# Autodesk Inventor assembly: GFRP_T2_05
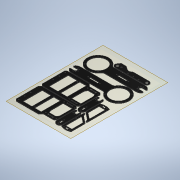
[picture p0: Inventor's stored thumbnail of the model, 180x180]
Saved by Autodesk Inventor 2020 (Build 240168000, 168)
## iProperties
Created: 2021-08-27
Part Number: GFRP_T2_05
Document SubType Name: Assembly
Designer: Masato
Author: Masato
## Documents named in this file (7)
- C:\Users\naoki\Documents\Inventor\CitBrains\git_clone\SUSTAINA_ver1_0\A_T2_175\SUSTAINA-OP\Cam\GFRP_T2_05.iam
- C:\Users\naoki\Documents\Inventor\CitBrains\git_clone\SUSTAINA_ver1_0\A_T2_175\SUSTAINA-OP\Cam\DisposableBoard.ipt
- C:\Users\naoki\Documents\Inventor\CitBrains\git_clone\SUSTAINA_ver1_0\A_T2_175\SUSTAINA-OP\UpperBody\Trunk\Trunk_upper_side_frame.ipt
- C:\Users\naoki\Documents\Inventor\CitBrains\git_clone\SUSTAINA_ver1_0\A_T2_175\SUSTAINA-OP\UpperBody\Arm\ForeArm_outside_frame.ipt
- C:\Users\naoki\Documents\Inventor\CitBrains\git_clone\SUSTAINA_ver1_0\A_T2_175\SUSTAINA-OP\UpperBody\Arm\UpperArm_side_frame.ipt
- C:\Users\naoki\Documents\Inventor\CitBrains\git_clone\SUSTAINA_ver1_0\A_T2_175\SUSTAINA-OP\UpperBody\Arm\ForeArm_inside_frame.ipt
- C:\Users\naoki\Documents\Inventor\CitBrains\git_clone\SUSTAINA_ver1_0\A_T2_175\SUSTAINA-OP\LowerBody\Link\BackLink_frame.ipt
## Components (10 placed, 6 different names)
1. DisposableBoard:1 — メイト:2, メイト:1, フラッシュ:1, フラッシュ:2, メイト:7, メイト:8, 正接:2, 正接:3, メイト:9, メイト:12, メイト:14, メイト:15, メイト:16, フラッシュ:3, フラッシュ:4, メイト:19, メイト:20, フラッシュ:6, 正接:6, 正接:7
2. Trunk_upper_side_frame:1 — メイト:15, フラッシュ:5, メイト:18, メイト:24, メイト:25
3. Trunk_upper_side_frame:2 — メイト:12, フラッシュ:3, フラッシュ:4, フラッシュ:5, メイト:18, メイト:21
4. ForeArm_outside_frame:1 — メイト:7, 正接:2, 正接:3, メイト:25, 正接:8, 正接:9
5. ForeArm_outside_frame:2 — メイト:8, メイト:17, 正接:7, 正接:8, 正接:9, 正接:10
6. UpperArm_side_frame:1 — メイト:9, メイト:23, 正接:4
7. ForeArm_inside_frame:1 — メイト:19, メイト:21, メイト:22, 正接:5, 正接:6
8. UpperArm_side_frame:2 — メイト:14, メイト:22, フラッシュ:6, 正接:4
9. ForeArm_inside_frame:2 — メイト:20, メイト:23, メイト:24, 正接:5
10. BackLink_frame:1 — メイト:16, メイト:17, 正接:10
## Relationships (33: Mate 18, Tangent 9, Flush 6)
- メイト:2 [Mate]: DisposableBoard:1
- メイト:1 [Mate]: DisposableBoard:1
- フラッシュ:1 [Flush]: DisposableBoard:1
- フラッシュ:2 [Flush]: DisposableBoard:1
- メイト:7 [Mate]: DisposableBoard:1 ↔ ForeArm_outside_frame:1
- メイト:8 [Mate]: DisposableBoard:1 ↔ ForeArm_outside_frame:2
- 正接:2 [Tangent] (2.5 mm): DisposableBoard:1 ↔ ForeArm_outside_frame:1
- 正接:3 [Tangent] (2.5 mm): DisposableBoard:1 ↔ ForeArm_outside_frame:1
- メイト:9 [Mate]: DisposableBoard:1 ↔ UpperArm_side_frame:1
- メイト:12 [Mate]: DisposableBoard:1 ↔ Trunk_upper_side_frame:2
- メイト:14 [Mate]: DisposableBoard:1 ↔ UpperArm_side_frame:2
- メイト:15 [Mate]: DisposableBoard:1 ↔ Trunk_upper_side_frame:1
- メイト:16 [Mate]: DisposableBoard:1 ↔ BackLink_frame:1
- メイト:17 [Mate] (3 mm): ForeArm_outside_frame:2 ↔ BackLink_frame:1
- フラッシュ:3 [Flush] (2 mm): DisposableBoard:1 ↔ Trunk_upper_side_frame:2
- フラッシュ:4 [Flush] (2 mm): DisposableBoard:1 ↔ Trunk_upper_side_frame:2
- フラッシュ:5 [Flush]: Trunk_upper_side_frame:1 ↔ Trunk_upper_side_frame:2
- メイト:18 [Mate] (2.5 mm): Trunk_upper_side_frame:1 ↔ Trunk_upper_side_frame:2
- メイト:19 [Mate]: DisposableBoard:1 ↔ ForeArm_inside_frame:1
- メイト:20 [Mate]: DisposableBoard:1 ↔ ForeArm_inside_frame:2
- メイト:21 [Mate] (2.5 mm): Trunk_upper_side_frame:2 ↔ ForeArm_inside_frame:1
- メイト:22 [Mate] (2.5 mm): ForeArm_inside_frame:1 ↔ UpperArm_side_frame:2
- メイト:23 [Mate] (2.5 mm): UpperArm_side_frame:1 ↔ ForeArm_inside_frame:2
- メイト:24 [Mate] (2.5 mm): Trunk_upper_side_frame:1 ↔ ForeArm_inside_frame:2
- フラッシュ:6 [Flush] (2 mm): DisposableBoard:1 ↔ UpperArm_side_frame:2
- 正接:4 [Tangent] (2.5 mm): UpperArm_side_frame:1 ↔ UpperArm_side_frame:2
- 正接:5 [Tangent] (2.5 mm): ForeArm_inside_frame:1 ↔ ForeArm_inside_frame:2
- メイト:25 [Mate] (2.5 mm): Trunk_upper_side_frame:1 ↔ ForeArm_outside_frame:1
- 正接:6 [Tangent] (2 mm): DisposableBoard:1 ↔ ForeArm_inside_frame:1
- 正接:7 [Tangent] (2 mm): DisposableBoard:1 ↔ ForeArm_outside_frame:2
- 正接:8 [Tangent] (2.5 mm): ForeArm_outside_frame:1 ↔ ForeArm_outside_frame:2
- 正接:9 [Tangent] (2.5 mm): ForeArm_outside_frame:1 ↔ ForeArm_outside_frame:2
- 正接:10 [Tangent] (2.5 mm): ForeArm_outside_frame:2 ↔ BackLink_frame:1
